# Autodesk Inventor assembly: MainAssembly
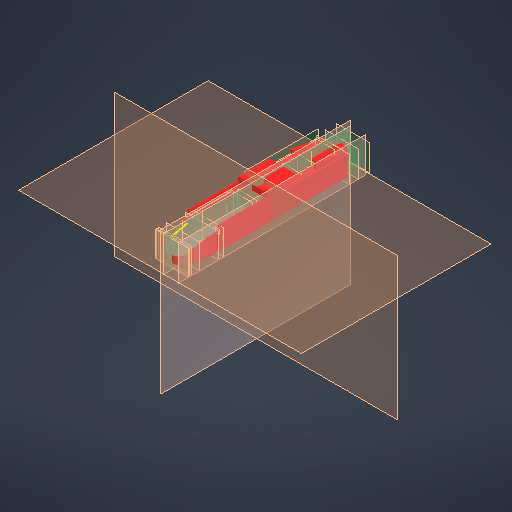
[picture p0: Inventor's stored thumbnail of the model, 512x512]
Saved by Autodesk Inventor 2027.1 (Build 311270010, 270A)
## iProperties
Created: 2026-09-14
Part Number: MainAssembly
Document SubType Name: Assembly
Designer: mateo
Author: mateo
## Documents named in this file (4)
- C:\Users\iqbal\OneDrive\Desktop\SWIFT_UAV\SWIFT-UAV\System_development\Pelican\structural_model\v0.3.1\MainAssembly\MainAssembly.iam
- C:\Users\iqbal\OneDrive\Desktop\SWIFT_UAV\SWIFT-UAV\System_development\Pelican\structural_model\v0.3.1\Parts\Fuselage\FuselageV2.ipt
- C:\Users\iqbal\OneDrive\Desktop\SWIFT_UAV\SWIFT-UAV\System_development\Pelican\structural_model\v0.3.1\Parts\Wings\WingBox.ipt
- C:\Users\iqbal\OneDrive\Desktop\SWIFT_UAV\SWIFT-UAV\System_development\Pelican\structural_model\v0.3.1\Parts\Aluminum_20x20\20x20x1295ExtrudedAluminum_MIR1.ipt
## Components (3 placed, 3 different names)
1. FuselageV2:1 — Mate:1, Mate:2, Mate:3, Mate:4, Mate:5, Mate:6
2. WingBox:1 — Mate:4, Mate:5, Mate:6, Mate:8, Mate:9
3. 20x20x1295ExtrudedAluminum_MIR1:1 — Mate:7, Mate:8, Mate:9
## Relationships (9: Mate 9)
- Mate:1: FuselageV2:1
- Mate:2 (-428.1297 mm): FuselageV2:1
- Mate:3: FuselageV2:1
- Mate:4: FuselageV2:1 ↔ WingBox:1
- Mate:5: FuselageV2:1 ↔ WingBox:1
- Mate:6: FuselageV2:1 ↔ WingBox:1
- Mate:7: 20x20x1295ExtrudedAluminum_MIR1:1
- Mate:8: WingBox:1 ↔ 20x20x1295ExtrudedAluminum_MIR1:1
- Mate:9: WingBox:1 ↔ 20x20x1295ExtrudedAluminum_MIR1:1
